# Autodesk Inventor assembly: Base Assembly
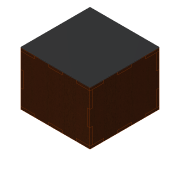
[picture p0: Inventor's stored thumbnail of the model, 180x180]
Saved by Autodesk Inventor 2016 (Build 200138000, 138)
## iProperties
Created: 2016-12-26
Part Number: Base Assembly
Document SubType Name: Conjunto soldado
Designer: Fernando
Weld Material: Aço macio soldado
Mass: 7265.04 g
Surface Area: 6091.54 cm^2
Volume: 2527.54 cm^3
Density: 2.87436 g/cm^3
SurfaceArea_m2: .61
Author: Fernando
## Documents named in this file (11)
- G:\00 - Files\00 - Personal\40 - Hobbies\90 - Projetos Particulares\40 - POV Display\01 - Mechanical Design\A03 - Base Assembly.iam
- G:\00 - Files\00 - Personal\40 - Hobbies\90 - Projetos Particulares\40 - POV Display\01 - Mechanical Design\P01 - Fan Motor.ipt
- G:\00 - Files\00 - Personal\40 - Hobbies\90 - Projetos Particulares\40 - POV Display\01 - Mechanical Design\M01 - Base Top.ipt
- G:\00 - Files\00 - Personal\40 - Hobbies\90 - Projetos Particulares\40 - POV Display\01 - Mechanical Design\M05 - Base Bottom.ipt
- G:\00 - Files\00 - Personal\40 - Hobbies\90 - Projetos Particulares\40 - POV Display\01 - Mechanical Design\M06 - Wall Side 1.ipt
- G:\00 - Files\00 - Personal\40 - Hobbies\90 - Projetos Particulares\40 - POV Display\01 - Mechanical Design\M07 - Wall Side 2.ipt
- G:\00 - Files\00 - Personal\40 - Hobbies\90 - Projetos Particulares\40 - POV Display\01 - Mechanical Design\M08 - Wall Side 3.ipt
- G:\00 - Files\00 - Personal\40 - Hobbies\90 - Projetos Particulares\40 - POV Display\01 - Mechanical Design\M09 - Wall Side 4.ipt
- G:\00 - Files\00 - Personal\40 - Hobbies\90 - Projetos Particulares\40 - POV Display\01 - Mechanical Design\M10 - Base Rubber.ipt
- G:\00 - Files\00 - Personal\40 - Hobbies\90 - Projetos Particulares\40 - POV Display\01 - Mechanical Design\P07 - M4 Bolt.ipt
- G:\00 - Files\00 - Personal\40 - Hobbies\90 - Projetos Particulares\40 - POV Display\01 - Mechanical Design\M15 - TX Coil.ipt
## Components (13 placed, 10 different names)
1. P01 - Fan Motor:1 — Insert:1
2. M01 - Base Top:2 — Insert:1, Mate:1, Flush:1, Mate:2, Mate:5, Flush:3, Mate:7, Flush:4, Mate:8, Flush:6, Flush:7, Insert:2, Insert:3, Insert:4, Insert:5, Insert:6
3. M05 - Base Bottom:1 — Mate:3, Flush:2, Mate:4, Mate:9, Flush:9, Flush:10
4. M06 - Wall Side 1:1 — Mate:1, Flush:1, Mate:2, Mate:3, Flush:2, Mate:4, Mate:6
5. M07 - Wall Side 2:1 — Mate:5, Flush:3, Mate:6, Flush:5
6. M08 - Wall Side 3:1 — Flush:4, Mate:8, Flush:5, Flush:8
7. M09 - Wall Side 4:1 — Flush:6, Flush:7, Flush:8
8. M10 - Base Rubber:1 — Mate:9, Flush:9, Flush:10
9. P07 - M4 Bolt:1 — Insert:3
10. P07 - M4 Bolt:2 — Insert:5
11. P07 - M4 Bolt:3 — Insert:2
12. P07 - M4 Bolt:4 — Insert:4
13. M15 - TX Coil:1 — Insert:6
## Relationships (25: Flush 10, Mate 9, Insert 6)
- Insert:1: P01 - Fan Motor:1 ↔ M01 - Base Top:2
- Mate:1: M01 - Base Top:2 ↔ M06 - Wall Side 1:1
- Flush:1: M01 - Base Top:2 ↔ M06 - Wall Side 1:1
- Mate:2: M01 - Base Top:2 ↔ M06 - Wall Side 1:1
- Mate:3: M05 - Base Bottom:1 ↔ M06 - Wall Side 1:1
- Flush:2: M05 - Base Bottom:1 ↔ M06 - Wall Side 1:1
- Mate:4: M05 - Base Bottom:1 ↔ M06 - Wall Side 1:1
- Mate:5: M01 - Base Top:2 ↔ M07 - Wall Side 2:1
- Flush:3: M01 - Base Top:2 ↔ M07 - Wall Side 2:1
- Mate:6: M06 - Wall Side 1:1 ↔ M07 - Wall Side 2:1
- Mate:7: M01 - Base Top:2
- Flush:4: M01 - Base Top:2 ↔ M08 - Wall Side 3:1
- Mate:8: M01 - Base Top:2 ↔ M08 - Wall Side 3:1
- Flush:5: M07 - Wall Side 2:1 ↔ M08 - Wall Side 3:1
- Flush:6: M01 - Base Top:2 ↔ M09 - Wall Side 4:1
- Flush:7: M01 - Base Top:2 ↔ M09 - Wall Side 4:1
- Flush:8: M08 - Wall Side 3:1 ↔ M09 - Wall Side 4:1
- Mate:9: M05 - Base Bottom:1 ↔ M10 - Base Rubber:1
- Flush:9: M05 - Base Bottom:1 ↔ M10 - Base Rubber:1
- Flush:10: M05 - Base Bottom:1 ↔ M10 - Base Rubber:1
- Insert:2: M01 - Base Top:2 ↔ P07 - M4 Bolt:3
- Insert:3: M01 - Base Top:2 ↔ P07 - M4 Bolt:1
- Insert:4: M01 - Base Top:2 ↔ P07 - M4 Bolt:4
- Insert:5: M01 - Base Top:2 ↔ P07 - M4 Bolt:2
- Insert:6 (3 mm): M01 - Base Top:2 ↔ M15 - TX Coil:1
